# Autodesk Inventor assembly: controller
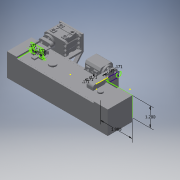
[picture p0: Inventor's stored thumbnail of the model, 180x180]
Saved by Autodesk Inventor 2016 SP1 (Build 200210100, 210)
## iProperties
Created: 2016-05-01
Part Number: controller
Document SubType Name: Assembly
Designer: Wes
Author: Wes
## Documents named in this file (7)
- C:\Users\Wes\Documents\School Stuff\ECE 499\final\inventor\controller.iam
- C:\Users\Wes\Documents\School Stuff\ECE 499\final\inventor\wiimote.ipt
- C:\Users\Wes\Documents\School Stuff\ECE 499\final\inventor\xl320Servo.ipt
- C:\Users\Wes\Documents\School Stuff\ECE 499\final\inventor\fire-bar.ipt
- C:\Users\Wes\Documents\School Stuff\ECE 499\final\inventor\dpad-bar.ipt
- C:\Users\Wes\Documents\School Stuff\ECE 499\final\inventor\cradle.ipt
- C:\Users\Wes\Documents\School Stuff\ECE 499\final\inventor\motor-mount-r.ipt
## Components (7 placed, 6 different names)
1. wiimote:1 — Angle:1, Flush:1, Mate:1, Mate:2, Mate:3, Mate:6, Mate:10, Mate:12, Mate:13, Mate:14, Mate:15, Mate:16, Mate:17
2. xl320Servo:1 — Mate:6, Mate:8, Mate:9, Mate:10, Mate:11, Rotational:1, Flush:2
3. xl320Servo:2 — Angle:1, Flush:1, Mate:1, Mate:2, Mate:4, Mate:5, Rotational:2
4. fire-bar:1 — Mate:3, Mate:4, Mate:5, Rotational:2
5. dpad-bar:1 — Mate:8, Mate:9, Mate:11, Rotational:1
6. cradle:1 — Mate:12, Mate:13, Mate:14, Mate:15, Mate:18
7. motor-mount-r:1 — Mate:16, Mate:17, Mate:18, Flush:2
## Relationships (22: Mate 17, Flush 2, RevoluteJoint 2, Angle 1)
- Angle:1 (0 deg): wiimote:1 ↔ xl320Servo:2
- Flush:1 (12.0904 mm): wiimote:1 ↔ xl320Servo:2
- Mate:1: wiimote:1 ↔ xl320Servo:2
- Mate:2 (5.08 mm): wiimote:1 ↔ xl320Servo:2
- Mate:3: wiimote:1 ↔ fire-bar:1
- Mate:4: xl320Servo:2 ↔ fire-bar:1
- Mate:5: xl320Servo:2 ↔ fire-bar:1
- Mate:6: wiimote:1 ↔ xl320Servo:1
- Mate:8: xl320Servo:1 ↔ dpad-bar:1
- Mate:9: xl320Servo:1 ↔ dpad-bar:1
- Mate:10: wiimote:1 ↔ xl320Servo:1
- Mate:11: xl320Servo:1 ↔ dpad-bar:1
- Mate:12: wiimote:1 ↔ cradle:1
- Mate:13: wiimote:1 ↔ cradle:1
- Mate:14: wiimote:1 ↔ cradle:1
- Mate:15: wiimote:1 ↔ cradle:1
- Mate:16: wiimote:1 ↔ motor-mount-r:1
- Mate:17: wiimote:1 ↔ motor-mount-r:1
- Mate:18: cradle:1 ↔ motor-mount-r:1
- Rotational:1 [RevoluteJoint] (17.272 mm): xl320Servo:1 ↔ dpad-bar:1
- Flush:2: xl320Servo:1 ↔ motor-mount-r:1
- Rotational:2 [RevoluteJoint]: xl320Servo:2 ↔ fire-bar:1
